# Autodesk Inventor assembly: Dedao_Mecanismo_Posição2
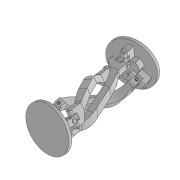
[picture p0: Inventor's stored thumbnail of the model, 180x180]
Saved by Autodesk Inventor 2020 (Build 240168000, 168)
## iProperties
Created: 2021-04-01
Part Number: Dedao_Mecanismo_Posição2
Document SubType Name: Assembly
Designer: deox
Author: deox
## Documents named in this file (5)
- C:\Users\deox\Desktop\TCC\Inventor Files\Dedo Kick\Dedao_Mecanismo_Posição2.iam
- C:\Users\deox\Desktop\TCC\Inventor Files\Dedo Kick\Base_Dedao.ipt
- C:\Users\deox\Desktop\TCC\Inventor Files\Dedo Kick\KNUCKLE_Dedao.ipt
- C:\Users\deox\Desktop\TCC\Inventor Files\Dedo Kick\LEG_Dedao.ipt
- C:\Users\deox\Desktop\TCC\Inventor Files\Dedo Kick\Pin_Dedao.ipt
## Components (23 placed, 4 different names)
1. Base_Dedao:1 — Mate:1, Mate:2, Mate:3, Mate:4, Mate:5, Mate:6, Mate:7, Mate:8, Mate:9, Mate:10, Mate:11, Mate:12, Angle:1
2. Base_Dedao:2 — Mate:25, Mate:26, Mate:27, Mate:28, Mate:29, Mate:30, Mate:31, Mate:32, Mate:33, Mate:34, Mate:35, Mate:36, Angle:1
3. KNUCKLE_Dedao:1 — Mate:9, Mate:10, Mate:13, Mate:14
4. KNUCKLE_Dedao:2 — Mate:1, Mate:2, Mate:17, Mate:18
5. KNUCKLE_Dedao:3 — Mate:5, Mate:6, Mate:21, Mate:22
6. KNUCKLE_Dedao:4 — Mate:27, Mate:28, Mate:39, Mate:40
7. KNUCKLE_Dedao:5 — Mate:25, Mate:26, Mate:37, Mate:38
8. KNUCKLE_Dedao:6 — Mate:29, Mate:30, Mate:41, Mate:42
9. LEG_Dedao:1 — Mate:13, Mate:14, Mate:15, Mate:16, Mate:37, Mate:38, Mate:47, Mate:48
10. LEG_Dedao:2 — Mate:17, Mate:18, Mate:19, Mate:20, Mate:41, Mate:42, Mate:43, Mate:44
11. LEG_Dedao:3 — Mate:21, Mate:22, Mate:23, Mate:24, Mate:39, Mate:40, Mate:45, Mate:46
12. Pin_Dedao:1 — Mate:3, Mate:4
13. Pin_Dedao:2 — Mate:11, Mate:12
14. Pin_Dedao:3 — Mate:7, Mate:8
15. Pin_Dedao:4 — Mate:19, Mate:20
16. Pin_Dedao:5 — Mate:15, Mate:16
17. Pin_Dedao:6 — Mate:23, Mate:24
18. Pin_Dedao:7 — Mate:35, Mate:36
19. Pin_Dedao:8 — Mate:33, Mate:34
20. Pin_Dedao:9 — Mate:31, Mate:32
21. Pin_Dedao:10 — Mate:43, Mate:44
22. Pin_Dedao:11 — Mate:47, Mate:48
23. Pin_Dedao:12 — Mate:45, Mate:46
## Relationships (49: Mate 48, Angle 1)
- Mate:1: Base_Dedao:1 ↔ KNUCKLE_Dedao:2
- Mate:2: Base_Dedao:1 ↔ KNUCKLE_Dedao:2
- Mate:3: Base_Dedao:1 ↔ Pin_Dedao:1
- Mate:4: Base_Dedao:1 ↔ Pin_Dedao:1
- Mate:5: Base_Dedao:1 ↔ KNUCKLE_Dedao:3
- Mate:6: Base_Dedao:1 ↔ KNUCKLE_Dedao:3
- Mate:7: Base_Dedao:1 ↔ Pin_Dedao:3
- Mate:8: Base_Dedao:1 ↔ Pin_Dedao:3
- Mate:9: Base_Dedao:1 ↔ KNUCKLE_Dedao:1
- Mate:10: Base_Dedao:1 ↔ KNUCKLE_Dedao:1
- Mate:11: Base_Dedao:1 ↔ Pin_Dedao:2
- Mate:12: Base_Dedao:1 ↔ Pin_Dedao:2
- Mate:13: KNUCKLE_Dedao:1 ↔ LEG_Dedao:1
- Mate:14: KNUCKLE_Dedao:1 ↔ LEG_Dedao:1
- Mate:15: LEG_Dedao:1 ↔ Pin_Dedao:5
- Mate:16: LEG_Dedao:1 ↔ Pin_Dedao:5
- Mate:17: KNUCKLE_Dedao:2 ↔ LEG_Dedao:2
- Mate:18: KNUCKLE_Dedao:2 ↔ LEG_Dedao:2
- Mate:19: LEG_Dedao:2 ↔ Pin_Dedao:4
- Mate:20: LEG_Dedao:2 ↔ Pin_Dedao:4
- Mate:21: KNUCKLE_Dedao:3 ↔ LEG_Dedao:3
- Mate:22: KNUCKLE_Dedao:3 ↔ LEG_Dedao:3
- Mate:23: LEG_Dedao:3 ↔ Pin_Dedao:6
- Mate:24: LEG_Dedao:3 ↔ Pin_Dedao:6
- Mate:25: Base_Dedao:2 ↔ KNUCKLE_Dedao:5
- Mate:26: Base_Dedao:2 ↔ KNUCKLE_Dedao:5
- Mate:27: Base_Dedao:2 ↔ KNUCKLE_Dedao:4
- Mate:28: Base_Dedao:2 ↔ KNUCKLE_Dedao:4
- Mate:29: Base_Dedao:2 ↔ KNUCKLE_Dedao:6
- Mate:30: Base_Dedao:2 ↔ KNUCKLE_Dedao:6
- Mate:31: Base_Dedao:2 ↔ Pin_Dedao:9
- Mate:32: Base_Dedao:2 ↔ Pin_Dedao:9
- Mate:33: Base_Dedao:2 ↔ Pin_Dedao:8
- Mate:34: Base_Dedao:2 ↔ Pin_Dedao:8
- Mate:35: Base_Dedao:2 ↔ Pin_Dedao:7
- Mate:36: Base_Dedao:2 ↔ Pin_Dedao:7
- Mate:37: KNUCKLE_Dedao:5 ↔ LEG_Dedao:1
- Mate:38: KNUCKLE_Dedao:5 ↔ LEG_Dedao:1
- Mate:39: KNUCKLE_Dedao:4 ↔ LEG_Dedao:3
- Mate:40: KNUCKLE_Dedao:4 ↔ LEG_Dedao:3
- Mate:41: KNUCKLE_Dedao:6 ↔ LEG_Dedao:2
- Mate:42: KNUCKLE_Dedao:6 ↔ LEG_Dedao:2
- Mate:43: LEG_Dedao:2 ↔ Pin_Dedao:10
- Mate:44: LEG_Dedao:2 ↔ Pin_Dedao:10
- Mate:45: LEG_Dedao:3 ↔ Pin_Dedao:12
- Mate:46: LEG_Dedao:3 ↔ Pin_Dedao:12
- Mate:47: LEG_Dedao:1 ↔ Pin_Dedao:11
- Mate:48: LEG_Dedao:1 ↔ Pin_Dedao:11
- Angle:1 (14 deg): Base_Dedao:1 ↔ Base_Dedao:2
